# Autodesk Inventor assembly: SPDT Toggle Switch
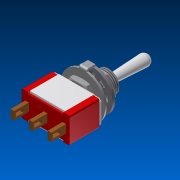
[picture p0: Inventor's stored thumbnail of the model, 180x180]
Saved by Autodesk Inventor 2011 SP1 (Build 150282100, 282)
## iProperties
Created: 2011-11-07
Part Number: SPDT Toggle Switch
Document SubType Name: Assembly
Designer: sdarley
Author: sdarley
## Documents named in this file (8)
- C:\Users\sdarley\Documents\Inventor\General Design Work\SPDT Toggle Switch\SPDT Toggle Switch.iam
- C:\Users\sdarley\Documents\Inventor\General Design Work\SPDT Toggle Switch\Components\SPDT Toggle Switch Base.ipt
- C:\Users\sdarley\Documents\Inventor\General Design Work\SPDT Toggle Switch\Components\SPDT Toggle Switch Pin.ipt
- C:\Users\sdarley\Documents\Inventor\General Design Work\SPDT Toggle Switch\Components\SPDT Toggle Switch Treaded Tube.ipt
- C:\Users\sdarley\Documents\Inventor\General Design Work\SPDT Toggle Switch\Components\Toggle Switch.ipt
- C:\Users\sdarley\Documents\Inventor\General Design Work\SPDT Toggle Switch\Components\M6x0.5 Hex Nut.ipt
- C:\Users\sdarley\Documents\Inventor\General Design Work\SPDT Toggle Switch\Components\SPDT Toggle Switch Anti-Rotation Washer.ipt
- C:\Users\sdarley\Documents\Inventor\Content Center Files\R2011\en-US\AS 1969(2)\AS 1969 - M6(2).ipt
## Components (10 placed, 7 different names)
1. SPDT Toggle Switch Base:1 — Flush:1, Flush:2, Mate:1, Mate:2, Flush:3, Flush:4, Flush:5, Flush:6, Flush:7, Flush:8
2. SPDT Toggle Switch Pin:1 — Flush:1, Flush:2
3. SPDT Toggle Switch Pin:2 — Mate:2, Flush:5, Flush:6
4. SPDT Toggle Switch Pin:3 — Mate:1, Flush:3, Flush:4
5. SPDT Toggle Switch Treaded Tube:1 — Flush:7, Flush:8, Mate:3, Mate:4, Insert:1, Mate:2, Mate:6
6. Toggle Switch:1 — Mate:3, Mate:4
7. M6x0.5 Hex Nut:1 — Insert:1, Flush:9
8. M6x0.5 Hex Nut:2 — Mate:6, Mate:7
9. SPDT Toggle Switch Anti-Rotation Washer:1 — Flush:9, Mate:5
10. AS 1969 (Internal Tooth Lock Washer Type A) M6:1 — Mate:2, Mate:5, Mate:7
## Relationships (18: Flush 9, Mate 8, Insert 1)
- Flush:1: SPDT Toggle Switch Base:1 ↔ SPDT Toggle Switch Pin:1
- Flush:2 (1 mm): SPDT Toggle Switch Base:1 ↔ SPDT Toggle Switch Pin:1
- Mate:1: SPDT Toggle Switch Base:1 ↔ SPDT Toggle Switch Pin:3
- Mate:2: SPDT Toggle Switch Base:1 ↔ SPDT Toggle Switch Pin:2
- Flush:3 (1 mm): SPDT Toggle Switch Base:1 ↔ SPDT Toggle Switch Pin:3
- Flush:4 (-2.4 mm): SPDT Toggle Switch Base:1 ↔ SPDT Toggle Switch Pin:3
- Flush:5 (2.4 mm): SPDT Toggle Switch Base:1 ↔ SPDT Toggle Switch Pin:2
- Flush:6 (6.025 mm): SPDT Toggle Switch Base:1 ↔ SPDT Toggle Switch Pin:2
- Flush:7: SPDT Toggle Switch Base:1 ↔ SPDT Toggle Switch Treaded Tube:1
- Flush:8: SPDT Toggle Switch Base:1 ↔ SPDT Toggle Switch Treaded Tube:1
- Mate:3: SPDT Toggle Switch Treaded Tube:1 ↔ Toggle Switch:1
- Mate:4 (9.5 mm): SPDT Toggle Switch Treaded Tube:1 ↔ Toggle Switch:1
- Insert:1: SPDT Toggle Switch Treaded Tube:1 ↔ M6x0.5 Hex Nut:1
- Flush:9: M6x0.5 Hex Nut:1 ↔ SPDT Toggle Switch Anti-Rotation Washer:1
- Mate:2: SPDT Toggle Switch Treaded Tube:1 ↔ AS 1969 (Internal Tooth Lock Washer Type A) M6:1
- Mate:5 (2 mm): SPDT Toggle Switch Anti-Rotation Washer:1 ↔ AS 1969 (Internal Tooth Lock Washer Type A) M6:1
- Mate:6: SPDT Toggle Switch Treaded Tube:1 ↔ M6x0.5 Hex Nut:2
- Mate:7: M6x0.5 Hex Nut:2 ↔ AS 1969 (Internal Tooth Lock Washer Type A) M6:1
